# Autodesk Inventor assembly: AX12
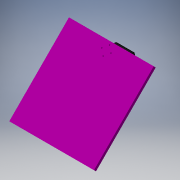
[picture p0: Inventor's stored thumbnail of the model, 180x180]
Saved by Autodesk Inventor 2017 (Build 210142000, 142)
## iProperties
Created: 2010-02-01
Part Number: AX12
Document SubType Name: Assembly
Designer: Andrew
Translation Standard: STEP AP203
File Name: AX12_Fixed.STEP
Preprocessor: SolidWorks 2010
Postprocessor: Build: 254, Release: 2008 - Date: Fri 03/23/2007
Sent Units: MILLIMETERS
Uncertainty: 1e-05
Author: Andrew
## Documents named in this file (7)
- C:\Users\franc\Desktop\EsialRobotik\Mecanique\robot-2017\AX12-minerai\AX12.iam
- C:\Users\franc\Desktop\EsialRobotik\Mecanique\robot-2017\AX12-minerai\ax12_wheel.ipt
- C:\Users\franc\Desktop\EsialRobotik\Mecanique\robot-2017\AX12-minerai\ax12_box.ipt
- C:\Users\franc\Desktop\EsialRobotik\Mecanique\robot-2017\AX12-minerai\ax12_cog.ipt
- C:\Users\franc\Desktop\EsialRobotik\Mecanique\robot-2017\AX12-minerai\plaque.ipt
- C:\Users\franc\Desktop\EsialRobotik\Mecanique\robot-2017\AX12-minerai\F2.ipt
- C:\Users\franc\Desktop\EsialRobotik\Mecanique\robot-2017\AX12-minerai\F3.ipt
## Components (6 placed, 6 different names)
1. ax12_wheel:1 — Insert:1, Mate:1, Mate:2, Mate:3
2. ax12_box:1 — Insert:1, Mate:7, Mate:8, Mate:9
3. ax12_cog:1
4. plaque:1 — Mate:4, Mate:5, Mate:6
5. F2:1 — Mate:1, Mate:2, Mate:3, Mate:4, Mate:5, Mate:6
6. F3:1 — Mate:7, Mate:8, Mate:9
## Relationships (10: Mate 9, Insert 1)
- Insert:1: ax12_wheel:1 ↔ ax12_box:1
- Mate:1: ax12_wheel:1 ↔ F2:1
- Mate:2: ax12_wheel:1 ↔ F2:1
- Mate:3: ax12_wheel:1 ↔ F2:1
- Mate:4: plaque:1 ↔ F2:1
- Mate:5: plaque:1 ↔ F2:1
- Mate:6: plaque:1 ↔ F2:1
- Mate:7: ax12_box:1 ↔ F3:1
- Mate:8: ax12_box:1 ↔ F3:1
- Mate:9: ax12_box:1 ↔ F3:1
